# Autodesk Inventor assembly: Car_Assembly
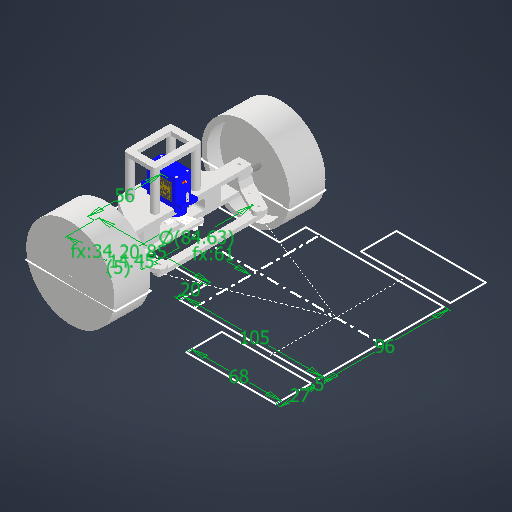
[picture p0: Inventor's stored thumbnail of the model, 512x512]
Saved by Autodesk Inventor 2025 (Build 290162010, 162A)
## iProperties
Created: 2024-05-24
Part Number: Car_Assembly
Document SubType Name: Assembly
Designer: Garfieldcmix
Author: Garfieldcmix
## Documents named in this file (10)
- C:\Users\chaya\Downloads\Inventor\Inventor\Car_Assembly.iam
- C:\Users\chaya\Documents\Inventor\SG90 - Micro Servo 9g - Tower Pro\SG90 - Micro Servo 9g - Tower Pro.iam
- C:\Users\chaya\Downloads\Inventor\Inventor\Front_Bridge.ipt
- C:\Users\chaya\Documents\Inventor\SG90 - Micro Servo 9g - Tower Pro\SG90 - Micro Servo 9g - Tower Pro.2.ipt
- C:\Users\chaya\Downloads\Inventor\Inventor\Front_Wheel_Anchor.ipt
- C:\Users\chaya\Downloads\Inventor\Inventor\Steering_Servo_Linkage.ipt
- C:\Users\chaya\Downloads\Inventor\Inventor\Front_Wheel_Anchor_MIR.ipt
- C:\Users\chaya\Downloads\Inventor\Inventor\Steering_Linkage.ipt
- C:\Users\chaya\Downloads\Inventor\Inventor\Wheel.ipt
- C:\Users\chaya\Downloads\Inventor\Inventor\Wheel_MIR.ipt
## Components (9 placed, 9 different names)
1. SG90_Servo [sub-assembly] — Mate:1, Mate:2
2. Servo_Arm — Mate:1, Mate:2, Flush:1, Mate:5, Mate:8
3. Front_Bridge:1 — Mate:3, Mate:4, Mate:5, Mate:9, Mate:10, Angle:1, Angle:2
4. Front_Left_Wheel_Anchor — Mate:3, Mate:4, Flush:1, Mate:6, Mate:7, Mate:11, Mate:12, Mate:14, Flush:2, Angle:1
5. Steering_Servo_Linkage:1 — Mate:6, Mate:7, Mate:8
6. Front_Right_Wheel_Anchor — Mate:9, Mate:10, Mate:13, Mate:15, Flush:3, Angle:2
7. Steering_Linkage:1 — Mate:11, Mate:12, Mate:13
8. Left_Front_Wheel — Mate:14, Flush:2
9. Right_Front_Wheel — Mate:15, Flush:3
## Relationships (20: Mate 15, Flush 3, Angle 2)
- Mate:1: SG90_Servo ↔ Servo_Arm
- Mate:2: SG90_Servo ↔ Servo_Arm
- Mate:3: Front_Bridge:1 ↔ Front_Left_Wheel_Anchor
- Mate:4: Front_Bridge:1 ↔ Front_Left_Wheel_Anchor
- Flush:1: Servo_Arm ↔ Front_Left_Wheel_Anchor
- Mate:5: Servo_Arm ↔ Front_Bridge:1
- Mate:6: Front_Left_Wheel_Anchor ↔ Steering_Servo_Linkage:1
- Mate:7: Front_Left_Wheel_Anchor ↔ Steering_Servo_Linkage:1
- Mate:8: Servo_Arm ↔ Steering_Servo_Linkage:1
- Mate:9: Front_Bridge:1 ↔ Front_Right_Wheel_Anchor
- Mate:10: Front_Bridge:1 ↔ Front_Right_Wheel_Anchor
- Mate:11: Front_Left_Wheel_Anchor ↔ Steering_Linkage:1
- Mate:12: Front_Left_Wheel_Anchor ↔ Steering_Linkage:1
- Mate:13: Front_Right_Wheel_Anchor ↔ Steering_Linkage:1
- Mate:14: Front_Left_Wheel_Anchor ↔ Left_Front_Wheel
- Flush:2: Front_Left_Wheel_Anchor ↔ Left_Front_Wheel
- Mate:15: Front_Right_Wheel_Anchor ↔ Right_Front_Wheel
- Flush:3: Front_Right_Wheel_Anchor ↔ Right_Front_Wheel
- Angle:1 (125 deg): Front_Bridge:1 ↔ Front_Left_Wheel_Anchor
- Angle:2 (-55 deg): Front_Bridge:1 ↔ Front_Right_Wheel_Anchor
